# Autodesk Inventor assembly: assembly
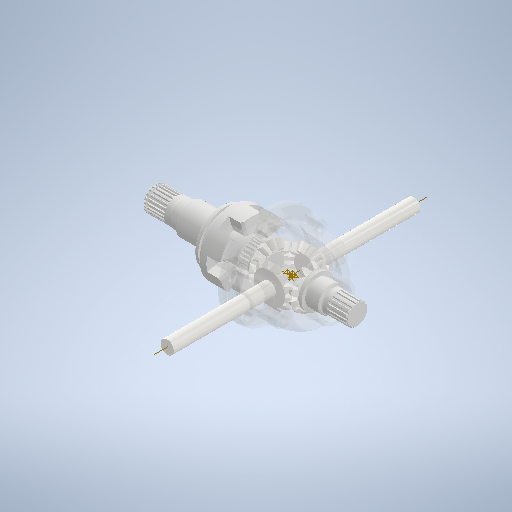
[picture p0: Inventor's stored thumbnail of the model, 512x512]
Saved by Autodesk Inventor 2025.2 (Build 292293000, 293)
## iProperties
Created: 2025-06-12
Part Number: assembly
Document SubType Name: Assembly
Designer: Kacper
Author: Kacper
## Documents named in this file (9)
- D:\studia\semestr 4\Grafika inżynierska\Projekt 4\mechanizm_rożnicowy.iam
- D:\studia\semestr 4\Grafika inżynierska\Projekt 4\housing.ipt
- D:\studia\semestr 4\Grafika inżynierska\Projekt 4\spacer_washer.ipt
- D:\studia\semestr 4\Grafika inżynierska\Projekt 4\rear_cover.ipt
- D:\studia\semestr 4\Grafika inżynierska\Projekt 4\bevel_gear_2.ipt
- D:\studia\semestr 4\Grafika inżynierska\Projekt 4\bevel_gear_1.ipt
- D:\studia\semestr 4\Grafika inżynierska\Projekt 4\shaft.ipt
- D:\studia\semestr 4\Grafika inżynierska\Projekt 4\shaft_fixture.ipt
- D:\studia\semestr 4\Grafika inżynierska\Projekt 4\bevel_gear_long.ipt
## Components (9 placed, 8 different names)
1. housing:1 — Mate:1, Mate:4, Mate:5, Mate:6, Mate:14, Mate:15, Mate:16, Mate:17, Mate:18
2. bevel_gear_2:1 — Mate:1, Mate:2, Mate:3, Rotation:1
3. spacer_washer:1 — Mate:2, Mate:3, Mate:4
4. rear_cover:1 — Mate:5, Mate:6, Mate:7, Mate:8, Mate:9, Mate:12, Mate:13, Mate:15
5. bevel_gear_1:1 — Mate:7, Mate:8, Flush:1, Mate:10
6. shaft:1 — Flush:1, Mate:9, Mate:10, Mate:11, Rotation:2, Rotation:4, Mate:19, Mate:21
7. shaft_fixture:1 — Mate:11, Mate:12, Mate:13
8. Bevel Gear2:1 — Mate:14, Mate:16, Rotation:1, Rotation:2
9. Bevel Gear2:2 — Mate:17, Mate:18, Rotation:4
## Relationships (26: Mate 21, RelateRotation 3, Flush 1, Angle 1)
- Mate:1: housing:1 ↔ bevel_gear_2:1
- Mate:2: bevel_gear_2:1 ↔ spacer_washer:1
- Mate:3: bevel_gear_2:1 ↔ spacer_washer:1
- Mate:4: housing:1 ↔ spacer_washer:1
- Mate:5: housing:1 ↔ rear_cover:1
- Mate:6: housing:1 ↔ rear_cover:1
- Mate:7: rear_cover:1 ↔ bevel_gear_1:1
- Mate:8: rear_cover:1 ↔ bevel_gear_1:1
- Flush:1 (-1 mm): bevel_gear_1:1 ↔ shaft:1
- Mate:9: rear_cover:1 ↔ shaft:1
- Mate:10: bevel_gear_1:1 ↔ shaft:1
- Mate:11: shaft:1 ↔ shaft_fixture:1
- Mate:12: rear_cover:1 ↔ shaft_fixture:1
- Mate:13: rear_cover:1 ↔ shaft_fixture:1
- Mate:14: housing:1 ↔ Bevel Gear2:1
- Mate:15: housing:1 ↔ rear_cover:1
- Mate:16 (7.5 mm): housing:1 ↔ Bevel Gear2:1
- Rotation:1 [RelateRotation] (0.9231 ul): bevel_gear_2:1 ↔ Bevel Gear2:1
- Rotation:2 [RelateRotation] (0.9231 ul): shaft:1 ↔ Bevel Gear2:1
- Mate:17: housing:1 ↔ Bevel Gear2:2
- Mate:18 (7.5 mm): housing:1 ↔ Bevel Gear2:2
- Rotation:4 [RelateRotation] (0.9231 ul): shaft:1 ↔ Bevel Gear2:2
- Mate:19: shaft:1
- Mate:20
- Mate:21: shaft:1
- Angle:1 (0 deg)
